# Autodesk Inventor assembly: Storage System Assembly
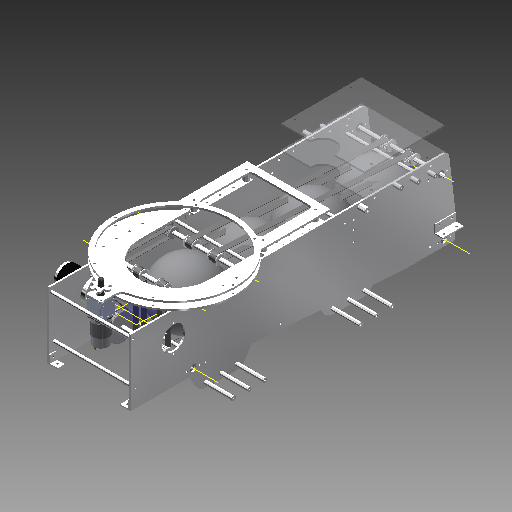
[picture p0: Inventor's stored thumbnail of the model, 512x512]
Saved by Autodesk Inventor 2019.4 (Build 234330000, 330)
## iProperties
Created: 2020-01-24
Part Number: Storage System Assembly
Document SubType Name: Assembly
Designer: admin
Mass: 10308.5 g
Surface Area: 22716.3 cm^2
Volume: 15823.1 cm^3
Density: 0.651483 g/cm^3
Author: admin
## Documents named in this file (31)
- C:\Users\admin\Desktop\FRC 2020 Engineering\GitHub\7738-2020\Robot V2\Storage System\Storage System Assembly.iam
- C:\Users\admin\Desktop\FRC 2020 Engineering\GitHub\7738-2020\Robot V2\Storage System\Storage Side Plate.ipt
- C:\Users\admin\Desktop\FRC 2020 Engineering\GitHub\7738-2020\Robot V2\Storage System\Storage System Assembly\Design Accelerator\Synchronous Belts Transmission1.iam
- C:\Users\admin\Desktop\FRC 2020 Engineering\GitHub\7738-2020\Robot V2\Storage System\Storage System Assembly\Design Accelerator\Synchronous Belts Transmission3.iam
- C:\Users\admin\Desktop\FRC 2020 Engineering\GitHub\7738-2020\Robot V2\Storage System\Storage System Assembly\Design Accelerator\Synchronous Belts Transmission4.iam
- C:\Users\admin\Desktop\FRC 2020 Engineering\GitHub\7738-2020\Robot V2\Storage System\Storage System Assembly\Design Accelerator\Synchronous Belts Transmission5.iam
- C:\Users\admin\Desktop\FRC 2020 Engineering\GitHub\7738-2020\Robot V2\Storage System\Storage System Assembly\Design Accelerator\Synchronous Belts Transmission6.iam
- C:\Users\admin\Desktop\FRC 2020 Engineering\GitHub\7738-2020\Power Cell.ipt
- C:\Users\admin\Desktop\FRC 2020 Engineering\GitHub\7738-2020\Robot V2\Storage System\Turret Support 2.ipt
- C:\Users\admin\Desktop\FRC 2020 Engineering\GitHub\7738-2020\Robot V2\Storage System\Turret Support.ipt
- C:\Users\admin\Desktop\FRC 2020 Engineering\GitHub\7738-2020\Robot V2\Storage System\Mounting Bracket.ipt
- C:\Users\admin\Desktop\FRC 2020 Engineering\GitHub\7738-2020\Robot V2\Storage System\Mounting Bracket 2.ipt
- C:\Users\admin\Desktop\FRC 2020 Engineering\GitHub\7738-2020\Robot V2\Storage System\Storage Plate Spacer.ipt
- C:\Users\admin\Desktop\FRC 2020 Engineering\GitHub\7738-2020\Robot V2\Storage System\Turret Bracket.ipt
- C:\Users\admin\Desktop\FRC 2020 Engineering\GitHub\7738-2020\Robot V2\Storage System\Small Support.ipt
- C:\Users\admin\Desktop\FRC 2020 Engineering\GitHub\7738-2020\Robot V2\Turret\Storage mounting spacers.ipt
- C:\Users\admin\Desktop\FRC 2020 Engineering\GitHub\7738-2020\Upper Stage\KFL08.ipt
- C:\Users\admin\Desktop\FRC 2020 Engineering\GitHub\7738-2020\Robot V2\Storage System\Turret Bracket 2.ipt
- C:\Users\admin\Desktop\FRC 2020 Engineering\GitHub\7738-2020\Robot V2\Storage System\Storage Axle.ipt
- C:\Users\admin\Desktop\FRC 2020 Engineering\GitHub\7738-2020\Robot V2\Storage System\Mini_CIM_Motor_217-3371.ipt
- C:\Users\admin\Desktop\FRC 2020 Engineering\GitHub\7738-2020\Robot V2\Storage System\Storage System Assembly\Design Accelerator\Synchronous Belts Transmission2.iam
- C:\Users\admin\Desktop\FRC 2020 Engineering\GitHub\7738-2020\Robot V2\Storage System\Motor Mount.ipt
- C:\Users\admin\Desktop\FRC 2020 Engineering\GitHub\7738-2020\Robot V2\Storage System\Motor Spacer.ipt
- C:\Users\admin\Desktop\FRC 2020 Engineering\GitHub\7738-2020\Robot V2\Storage System\Storage System Assembly\Design Accelerator\Synchronous Belts Transmission7.iam
- C:\Users\admin\Desktop\FRC 2020 Engineering\GitHub\7738-2020\Elevator MK2\Wood Electronic  1.ipt
- C:\Users\admin\Desktop\FRC 2020 Engineering\GitHub\7738-2020\Robot V2\Storage System\Turret Drive Gear.ipt
- C:\Users\admin\Desktop\FRC 2020 Engineering\GitHub\7738-2020\Robot V2\VexVersa.iam
- C:\Users\admin\Desktop\FRC 2020 Engineering\GitHub\7738-2020\Robot V2\Turret\F6800.ipt
- C:\Users\admin\Desktop\FRC 2020 Engineering\GitHub\7738-2020\Robot V2\Storage System\Storage Axle Intake.ipt
- C:\Users\admin\Desktop\FRC 2020 Engineering\GitHub\7738-2020\Robot V2\Intake V2\Pneumatic Spcaer 2.ipt
- C:\Users\admin\Desktop\FRC 2020 Engineering\GitHub\7738-2020\Cover Spacer.ipt
## Components (77 placed, 24 different names)
1. Storage Side Plate:1 — Mate:3, Flush:2, Mate:43, Flush:7, Mate:44, Mate:45, Mate:46, Mate:47, Mate:48, Mate:50, Mate:51, Mate:52, Mate:92, Flush:17, Mate:108, Mate:109, Mate:110, Mate:111, Mate:112, Mate:113, Mate:114, Mate:115, Mate:116, Mate:117, Mate:118, Mate:119, Mate:148, Flush:19, Flush:20, Mate:151, Flush:21, Mate:185, Mate:188, Mate:189, Mate:190, Mate:191, Mate:196, Mate:197, Mate:203, Mate:204, Flush:34, Flush:35, Mate:224, Mate:235, Flush:37, Flush:38, Mate:237, Flush:40, Mate:246, Mate:247, Mate:248, Mate:253, Mate:254, Mate:258, Mate:259, Mate:260, Mate:261, Mate:262, Mate:263, Mate:264, Mate:265
2. Synchronous Belts Transmission:1 [sub-assembly]
3. Synchronous Belts Transmission:2 [sub-assembly]
4. Synchronous Belts Transmission:3 [sub-assembly] — Symmetry:1
5. Synchronous Belts Transmission:4 [sub-assembly] — Symmetry:1
6. Synchronous Belts Transmission:5 [sub-assembly]
7. Power Cell:1 — Mate:4, Mate:231
8. Power Cell:2 — Mate:5, Mate:234
9. Power Cell:3 — Mate:6, Mate:232
10. Power Cell:4 — Mate:7, Mate:233
11. Mounting Bracket 2:1 — Mate:223, Flush:32, Flush:33
12. Mounting Bracket 2:2 — Mate:43, Flush:7, Flush:34, Flush:35
13. Storage Plate Spacer:1 — Mate:46
14. Storage Plate Spacer:2 — Mate:48
15. Storage Plate Spacer:3 — Mate:44
16. Storage Plate Spacer:4 — Mate:51
17. Storage Plate Spacer:5 — Mate:47
18. Storage Plate Spacer:6 — Mate:50, Mate:224
19. Storage Plate Spacer:8 — Mate:52
20. Storage Plate Spacer:9 — Mate:45
21. Turret Bracket:2 — Flush:25, Mate:169, Flush:26
22. Small Support:1 — Mate:104, Mate:107
23. Small Support:2 — Mate:102, Mate:103
24. Small Support:3 — Mate:105, Mate:106
25. Small Support:4 — Mate:99, Mate:100, Mate:101
26. Turret Bracket:5 — Mate:92, Flush:17, Mate:98, Mate:100, Mate:103, Flush:26, Mate:238
27. Turret Support 2:2 — Mate:98, Mate:99, Mate:101, Mate:102, Mate:104, Mate:105, Mate:106, Mate:107, Mate:241, Mate:242, Flush:43
28. Storage mounting spacers:1 — Mate:108, Mate:119
29. Storage mounting spacers:2 — Mate:109, Mate:118
30. Storage mounting spacers:3 — Mate:110, Mate:117
31. Storage mounting spacers:4 — Mate:111, Mate:114
32. Storage mounting spacers:5 — Mate:112, Mate:115
33. Storage mounting spacers:6 — Mate:113, Mate:116
34. Storage mounting spacers:7 — Mate:155, Mate:161
35. Storage mounting spacers:8 — Mate:156, Mate:162
36. Storage mounting spacers:9 — Mate:157, Mate:163
37. Storage mounting spacers:10 — Mate:159, Mate:165
38. Storage mounting spacers:11 — Mate:158, Mate:164
39. Storage mounting spacers:12 — Mate:160, Mate:166
40. KFL08:2 — Mate:178, Mate:179, Mate:180, Mate:206
41. KFL08:3 — Mate:182, Mate:183, Mate:184, Mate:209
42. KFL08:4 — Mate:176, Mate:177, Mate:181, Mate:205
43. Turret Bracket 2:1 — Mate:152, Flush:22
44. Turret Bracket 2:2 — Mate:148, Flush:19
45. Turret Support:4 — Mate:149, Mate:150, Mate:154
46. Storage Side Plate:2 — Flush:20, Mate:151, Flush:21, Mate:152, Flush:22, Mate:154, Mate:155, Mate:156, Mate:157, Mate:158, Mate:159, Mate:160, Mate:161, Mate:162, Mate:163, Mate:164, Mate:165, Mate:166, Flush:25, Mate:169, Mate:176, Mate:177, Mate:178, Mate:179, Mate:180, Mate:181, Mate:182, Mate:183, Mate:184, Flush:27, Mate:214, Mate:215, Mate:216, Mate:223, Flush:32, Flush:33, Mate:236, Flush:36, Flush:39, Mate:244, Mate:245, Mate:249, Mate:252, Mate:255, Mate:266, Mate:267, Mate:268, Mate:269, Mate:270, Mate:271
47. KFL08:6 — Mate:188, Mate:196, Mate:197, Mate:200
48. KFL08:7 — Mate:189, Mate:190, Mate:191, Mate:202
49. KFL08:8 — Mate:185, Mate:201, Mate:203, Mate:204
50. Storage Axle:1 — Mate:202, Mate:206
51. Storage Axle:2 — Mate:201, Mate:205
52. Storage Axle:3 — Mate:200, Mate:209
53. Mini_CIM_Motor_217-3371:1 — Mate:210, Flush:27, Mate:211, Mate:212, Mate:213
54. Synchronous Belts Transmission:6 [sub-assembly] — Mate:210
55. Motor Mount:1 — Mate:211, Mate:212, Mate:213, Mate:214, Mate:217, Mate:218
56. Motor Spacer:1 — Mate:215, Mate:218
57. Motor Spacer:2 — Mate:216, Mate:217
58. Synchronous Belts Transmission:7 [sub-assembly]
59. Mounting Bracket:1 — Mate:235, Flush:37, Flush:38
60. Mounting Bracket:2 — Mate:236, Flush:36, Flush:39
61. Wood Electronic  1:1 — Mate:237, Flush:40, Mate:238, Mate:239, Flush:41, Flush:42
62. Wood Electronic  1:2 — Mate:239, Flush:41, Flush:42
63. Turret Drive Gear:2 — Mate:241, Mate:243
64. VexVersa:1 [sub-assembly] — Mate:242, Flush:43, Mate:243
65. KFL08:9 — Mate:244, Mate:245, Mate:249, Mate:250
66. KFL08:10 — Mate:246, Mate:247, Mate:248, Mate:251
67. Storage Axle:4 — Mate:250, Mate:251
68. F6800:1 — Mate:252, Mate:255, Mate:256, Mate:257
69. F6800:2 — Mate:253, Mate:254
70. Storage Axle Intake:1 — Mate:256, Mate:257
71. Pneumatic Spcaer 2:1 — Mate:258, Mate:259
72. Cover Spacer:1 — Mate:260, Mate:263
73. Cover Spacer:2 — Mate:261, Mate:264
74. Cover Spacer:3 — Mate:262, Mate:265
75. Cover Spacer:4 — Mate:268, Mate:271
76. Cover Spacer:5 — Mate:266, Mate:269
77. Cover Spacer:6 — Mate:267, Mate:270
## Relationships (154: Mate 131, Flush 22, Symmetry 1)
- Mate:3 (114.3 mm): Storage Side Plate:1
- Mate:4: Power Cell:1
- Mate:5: Power Cell:2
- Mate:6: Power Cell:3
- Mate:7: Power Cell:4
- Flush:2: Storage Side Plate:1
- Mate:43: Storage Side Plate:1 ↔ Mounting Bracket 2:2
- Flush:7: Storage Side Plate:1 ↔ Mounting Bracket 2:2
- Mate:44: Storage Side Plate:1 ↔ Storage Plate Spacer:3
- Mate:45: Storage Side Plate:1 ↔ Storage Plate Spacer:9
- Mate:46: Storage Side Plate:1 ↔ Storage Plate Spacer:1
- Mate:47: Storage Side Plate:1 ↔ Storage Plate Spacer:5
- Mate:48: Storage Side Plate:1 ↔ Storage Plate Spacer:2
- Mate:50: Storage Side Plate:1 ↔ Storage Plate Spacer:6
- Mate:51: Storage Side Plate:1 ↔ Storage Plate Spacer:4
- Mate:52: Storage Side Plate:1 ↔ Storage Plate Spacer:8
- Mate:92: Storage Side Plate:1 ↔ Turret Bracket:5
- Flush:17: Storage Side Plate:1 ↔ Turret Bracket:5
- Mate:98: Turret Bracket:5 ↔ Turret Support 2:2
- Mate:99: Small Support:4 ↔ Turret Support 2:2
- Mate:100: Small Support:4 ↔ Turret Bracket:5
- Mate:101: Small Support:4 ↔ Turret Support 2:2
- Mate:102: Small Support:2 ↔ Turret Support 2:2
- Mate:103: Small Support:2 ↔ Turret Bracket:5
- Mate:104: Small Support:1 ↔ Turret Support 2:2
- Mate:105: Small Support:3 ↔ Turret Support 2:2
- Mate:106: Small Support:3 ↔ Turret Support 2:2
- Mate:107: Small Support:1 ↔ Turret Support 2:2
- Mate:108: Storage Side Plate:1 ↔ Storage mounting spacers:1
- Mate:109: Storage Side Plate:1 ↔ Storage mounting spacers:2
- Mate:110: Storage Side Plate:1 ↔ Storage mounting spacers:3
- Mate:111: Storage Side Plate:1 ↔ Storage mounting spacers:4
- Mate:112: Storage Side Plate:1 ↔ Storage mounting spacers:5
- Mate:113: Storage Side Plate:1 ↔ Storage mounting spacers:6
- Mate:114: Storage Side Plate:1 ↔ Storage mounting spacers:4
- Mate:115: Storage Side Plate:1 ↔ Storage mounting spacers:5
- Mate:116: Storage Side Plate:1 ↔ Storage mounting spacers:6
- Mate:117: Storage Side Plate:1 ↔ Storage mounting spacers:3
- Mate:118: Storage Side Plate:1 ↔ Storage mounting spacers:2
- Mate:119: Storage Side Plate:1 ↔ Storage mounting spacers:1
- Mate:148: Storage Side Plate:1 ↔ Turret Bracket 2:2
- Flush:19: Storage Side Plate:1 ↔ Turret Bracket 2:2
- Mate:149: Turret Support:4
- Mate:150: Turret Support:4
- Flush:20: Storage Side Plate:1 ↔ Storage Side Plate:2
- Mate:151 (228.6 mm): Storage Side Plate:1 ↔ Storage Side Plate:2
- Flush:21: Storage Side Plate:1 ↔ Storage Side Plate:2
- Mate:152: Turret Bracket 2:1 ↔ Storage Side Plate:2
- Flush:22: Turret Bracket 2:1 ↔ Storage Side Plate:2
- Mate:154: Turret Support:4 ↔ Storage Side Plate:2
- Mate:155: Storage mounting spacers:7 ↔ Storage Side Plate:2
- Mate:156: Storage mounting spacers:8 ↔ Storage Side Plate:2
- Mate:157: Storage mounting spacers:9 ↔ Storage Side Plate:2
- Mate:158: Storage mounting spacers:11 ↔ Storage Side Plate:2
- Mate:159: Storage mounting spacers:10 ↔ Storage Side Plate:2
- Mate:160: Storage mounting spacers:12 ↔ Storage Side Plate:2
- Mate:161: Storage mounting spacers:7 ↔ Storage Side Plate:2
- Mate:162: Storage mounting spacers:8 ↔ Storage Side Plate:2
- Mate:163: Storage mounting spacers:9 ↔ Storage Side Plate:2
- Mate:164: Storage mounting spacers:11 ↔ Storage Side Plate:2
- Mate:165: Storage mounting spacers:10 ↔ Storage Side Plate:2
- Mate:166: Storage mounting spacers:12 ↔ Storage Side Plate:2
- Flush:25: Turret Bracket:2 ↔ Storage Side Plate:2
- Mate:169: Turret Bracket:2 ↔ Storage Side Plate:2
- Flush:26: Turret Bracket:2 ↔ Turret Bracket:5
- Mate:176: KFL08:4 ↔ Storage Side Plate:2
- Mate:177: KFL08:4 ↔ Storage Side Plate:2
- Mate:178: KFL08:2 ↔ Storage Side Plate:2
- Mate:179: KFL08:2 ↔ Storage Side Plate:2
- Mate:180: KFL08:2 ↔ Storage Side Plate:2
- Mate:181: KFL08:4 ↔ Storage Side Plate:2
- Mate:182: KFL08:3 ↔ Storage Side Plate:2
- Mate:183: KFL08:3 ↔ Storage Side Plate:2
- Mate:184: KFL08:3 ↔ Storage Side Plate:2
- Mate:185: Storage Side Plate:1 ↔ KFL08:8
- Mate:188: Storage Side Plate:1 ↔ KFL08:6
- Mate:189: Storage Side Plate:1 ↔ KFL08:7
- Mate:190: Storage Side Plate:1 ↔ KFL08:7
- Mate:191: Storage Side Plate:1 ↔ KFL08:7
- Mate:196: Storage Side Plate:1 ↔ KFL08:6
- Mate:197: Storage Side Plate:1 ↔ KFL08:6
- Mate:200: KFL08:6 ↔ Storage Axle:3
- Mate:201: KFL08:8 ↔ Storage Axle:2
- Mate:202: KFL08:7 ↔ Storage Axle:1
- Mate:203: Storage Side Plate:1 ↔ KFL08:8
- Mate:204: Storage Side Plate:1 ↔ KFL08:8
- Mate:205: KFL08:4 ↔ Storage Axle:2
- Mate:206: KFL08:2 ↔ Storage Axle:1
- Mate:209: KFL08:3 ↔ Storage Axle:3
- Mate:210: Mini_CIM_Motor_217-3371:1 ↔ Synchronous Belts Transmission:6
- Flush:27 (-5 mm): Storage Side Plate:2 ↔ Mini_CIM_Motor_217-3371:1
- Mate:211: Mini_CIM_Motor_217-3371:1 ↔ Motor Mount:1
- Mate:212: Mini_CIM_Motor_217-3371:1 ↔ Motor Mount:1
- Mate:213: Mini_CIM_Motor_217-3371:1 ↔ Motor Mount:1
- Mate:214: Storage Side Plate:2 ↔ Motor Mount:1
- Mate:215: Storage Side Plate:2 ↔ Motor Spacer:1
- Mate:216: Storage Side Plate:2 ↔ Motor Spacer:2
- Mate:217: Motor Mount:1 ↔ Motor Spacer:2
- Mate:218: Motor Mount:1 ↔ Motor Spacer:1
- Mate:223: Mounting Bracket 2:1 ↔ Storage Side Plate:2
- Flush:32: Mounting Bracket 2:1 ↔ Storage Side Plate:2
- Flush:33: Mounting Bracket 2:1 ↔ Storage Side Plate:2
- Flush:34: Storage Side Plate:1 ↔ Mounting Bracket 2:2
- Flush:35: Storage Side Plate:1 ↔ Mounting Bracket 2:2
- Mate:224: Storage Side Plate:1 ↔ Storage Plate Spacer:6
- Symmetry:1: Synchronous Belts Transmission:3 ↔ Synchronous Belts Transmission:4
- Mate:231: Power Cell:1
- Mate:232: Power Cell:3
- Mate:233: Power Cell:4
- Mate:234: Power Cell:2
- Mate:235: Storage Side Plate:1 ↔ Mounting Bracket:1
- Mate:236: Storage Side Plate:2 ↔ Mounting Bracket:2
- Flush:36: Storage Side Plate:2 ↔ Mounting Bracket:2
- Flush:37: Storage Side Plate:1 ↔ Mounting Bracket:1
- Flush:38 (45 mm): Storage Side Plate:1 ↔ Mounting Bracket:1
- Flush:39 (45 mm): Storage Side Plate:2 ↔ Mounting Bracket:2
- Mate:237: Storage Side Plate:1 ↔ Wood Electronic  1:1
- Flush:40: Storage Side Plate:1 ↔ Wood Electronic  1:1
- Mate:238 (110 mm): Turret Bracket:5 ↔ Wood Electronic  1:1
- Mate:239 (60 mm): Wood Electronic  1:1 ↔ Wood Electronic  1:2
- Flush:41: Wood Electronic  1:1 ↔ Wood Electronic  1:2
- Flush:42: Wood Electronic  1:1 ↔ Wood Electronic  1:2
- Mate:241 (15 mm): Turret Support 2:2 ↔ Turret Drive Gear:2
- Mate:242: Turret Support 2:2 ↔ VexVersa:1
- Flush:43: Turret Support 2:2 ↔ VexVersa:1
- Mate:243: Turret Drive Gear:2 ↔ VexVersa:1
- Mate:244: Storage Side Plate:2 ↔ KFL08:9
- Mate:245: Storage Side Plate:2 ↔ KFL08:9
- Mate:246: Storage Side Plate:1 ↔ KFL08:10
- Mate:247: Storage Side Plate:1 ↔ KFL08:10
- Mate:248: Storage Side Plate:1 ↔ KFL08:10
- Mate:249: Storage Side Plate:2 ↔ KFL08:9
- Mate:250: KFL08:9 ↔ Storage Axle:4
- Mate:251: KFL08:10 ↔ Storage Axle:4
- Mate:252: Storage Side Plate:2 ↔ F6800:1
- Mate:253: Storage Side Plate:1 ↔ F6800:2
- Mate:254 (0.2 mm): Storage Side Plate:1 ↔ F6800:2
- Mate:255 (0.2 mm): Storage Side Plate:2 ↔ F6800:1
- Mate:256: F6800:1 ↔ Storage Axle Intake:1
- Mate:257: F6800:1 ↔ Storage Axle Intake:1
- Mate:258: Storage Side Plate:1 ↔ Pneumatic Spcaer 2:1
- Mate:259: Storage Side Plate:1 ↔ Pneumatic Spcaer 2:1
- Mate:260: Storage Side Plate:1 ↔ Cover Spacer:1
- Mate:261: Storage Side Plate:1 ↔ Cover Spacer:2
- Mate:262: Storage Side Plate:1 ↔ Cover Spacer:3
- Mate:263: Storage Side Plate:1 ↔ Cover Spacer:1
- Mate:264: Storage Side Plate:1 ↔ Cover Spacer:2
- Mate:265: Storage Side Plate:1 ↔ Cover Spacer:3
- Mate:266: Storage Side Plate:2 ↔ Cover Spacer:5
- Mate:267: Storage Side Plate:2 ↔ Cover Spacer:6
- Mate:268: Storage Side Plate:2 ↔ Cover Spacer:4
- Mate:269: Storage Side Plate:2 ↔ Cover Spacer:5
- Mate:270: Storage Side Plate:2 ↔ Cover Spacer:6
- Mate:271: Storage Side Plate:2 ↔ Cover Spacer:4
